# Autodesk Inventor assembly: リンク_6_1
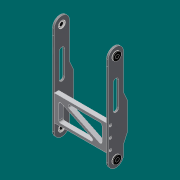
[picture p0: Inventor's stored thumbnail of the model, 180x180]
Saved by Autodesk Inventor 2016 (Build 200138000, 138)
## iProperties
Created: 2016-08-23
Part Number: リンク_6_1
Material: 一般
Document SubType Name: Assembly
Designer: hiro
Mass: 25.265 g
Surface Area: 146.992 cm^2
Volume: 11.3922 cm^3
Density: 2.21774 g/cm^3
Author: hiro
## Documents named in this file (5)
- C:\Users\hiro\Documents\kenkyuu\二足\二足ver6.0\下半身_160823\リンク\リンク_6_3.iam
- C:\Users\hiro\Documents\kenkyuu\二足\二足ver6.0\下半身\リンク\ふくらはぎ\リンク_ふくらはぎ_サブフレーム_1_2(予備案).ipt
- C:\Users\hiro\Documents\kenkyuu\二足\二足ver6.0\既製品\NSK_RB_MF85ZZ\MF85ZZ.iam
- C:\Users\hiro\Documents\kenkyuu\二足\二足ver6.0\既製品\新規購入\D4050-9120B.ipt
- C:\Users\hiro\Documents\kenkyuu\二足\二足ver6.0\下半身_160823\リンク\リンク_メインフレーム_6_1.ipt
## Components (11 placed, 4 different names)
1. リンク_ふくらはぎ_サブフレーム_1_2(予備案):1 — 挿入:25, 挿入:26, 挿入:27, 挿入:30, 挿入:31, 挿入:32
2. MF85ZZ:1 [sub-assembly] — 挿入:22, 挿入:34
3. MF85ZZ:2 [sub-assembly] — 挿入:24, 挿入:29
4. MF85ZZ:3 [sub-assembly] — 挿入:21, 挿入:33
5. MF85ZZ:4 [sub-assembly] — 挿入:23, 挿入:28
6. D4050-9120B:1 — 挿入:23
7. D4050-9120B:2 — 挿入:24
8. D4050-9120B:3 — 挿入:22
9. D4050-9120B:4 — 挿入:21
10. リンク_メインフレーム_6_1:1 — 挿入:30, 挿入:31, 挿入:32, 挿入:33, 挿入:34
11. リンク_メインフレーム_6_1:2 — 挿入:25, 挿入:26, 挿入:27, 挿入:28, 挿入:29
## Relationships (14: Insert 14)
- 挿入:21 [Insert]: MF85ZZ:3 ↔ D4050-9120B:4
- 挿入:22 [Insert]: MF85ZZ:1 ↔ D4050-9120B:3
- 挿入:23 [Insert]: MF85ZZ:4 ↔ D4050-9120B:1
- 挿入:24 [Insert]: MF85ZZ:2 ↔ D4050-9120B:2
- 挿入:25 [Insert]: リンク_ふくらはぎ_サブフレーム_1_2(予備案):1 ↔ リンク_メインフレーム_6_1:2
- 挿入:26 [Insert]: リンク_ふくらはぎ_サブフレーム_1_2(予備案):1 ↔ リンク_メインフレーム_6_1:2
- 挿入:27 [Insert]: リンク_ふくらはぎ_サブフレーム_1_2(予備案):1 ↔ リンク_メインフレーム_6_1:2
- 挿入:28 [Insert]: MF85ZZ:4 ↔ リンク_メインフレーム_6_1:2
- 挿入:29 [Insert]: MF85ZZ:2 ↔ リンク_メインフレーム_6_1:2
- 挿入:30 [Insert]: リンク_ふくらはぎ_サブフレーム_1_2(予備案):1 ↔ リンク_メインフレーム_6_1:1
- 挿入:31 [Insert]: リンク_ふくらはぎ_サブフレーム_1_2(予備案):1 ↔ リンク_メインフレーム_6_1:1
- 挿入:32 [Insert]: リンク_ふくらはぎ_サブフレーム_1_2(予備案):1 ↔ リンク_メインフレーム_6_1:1
- 挿入:33 [Insert]: MF85ZZ:3 ↔ リンク_メインフレーム_6_1:1
- 挿入:34 [Insert]: MF85ZZ:1 ↔ リンク_メインフレーム_6_1:1
